# Autodesk Inventor assembly: St
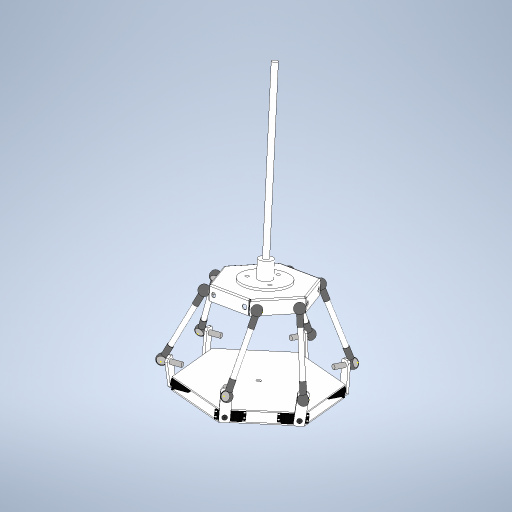
[picture p0: Inventor's stored thumbnail of the model, 512x512]
Saved by Autodesk Inventor 2023 (Build 270158000, 158)
## iProperties
Created: 2022-07-07
Part Number: St
Document SubType Name: Assembly
Designer: earls
Author: earls
## Documents named in this file (18)
- C:\Users\earls\Documents\stewart-platform\CAD\St.iam
- C:\Users\earls\Documents\stewart-platform\CAD\Bottom plate 2.5mm.ipt
- C:\Users\earls\Documents\stewart-platform\CAD\ServoMotor\Servo.ipt
- C:\Users\earls\Documents\stewart-platform\CAD\Servo arm.ipt
- C:\Users\earls\Documents\stewart-platform\CAD\Spherical joint\Part1.ipt
- C:\Users\earls\Documents\stewart-platform\CAD\Spherical joint\Part2.ipt
- C:\Users\earls\Documents\stewart-platform\CAD\Rod qty-6 Not hollow.ipt
- C:\Users\earls\Documents\stewart-platform\CAD\Moving platform.ipt
- C:\Users\earls\Documents\stewart-platform\CAD\Test flange.ipt
- C:\Users\earls\Documents\stewart-platform\CAD\Strut.ipt
- C:\Users\earls\Documents\stewart-platform\CAD\St\AIP\FEA\e0wa6g2m8.fins
- C:\Users\earls\Documents\stewart-platform\CAD\St\AIP\FEA\e0wa6g2m8.fsat
- C:\Users\earls\Documents\stewart-platform\CAD\St\AIP\FEA\e0wa6g2n4.ftes
- C:\Users\earls\Documents\stewart-platform\CAD\St\AIP\FEA\e0wa6g2n4.fwiz
- C:\Users\earls\Documents\stewart-platform\CAD\St\AIP\FEA\e0wa6g2u8.fmsh
- C:\Users\earls\Documents\stewart-platform\CAD\St\AIP\FEA\e0wa6g2v4.fres
- C:\Users\earls\Documents\stewart-platform\CAD\St\AIP\FEA\e0wa6g3cw.fmsh
- C:\Users\earls\Documents\stewart-platform\CAD\St\AIP\FEA\e0wa6g3cx.fres
## Components (47 placed, 9 different names)
1. Bottom plate 2.5mm:1 — Mate:4, Mate:5, Mate:6, Mate:7, Mate:8, Mate:9, Mate:10, Mate:11, Mate:12, Mate:13, Mate:14, Mate:15, Mate:16, Mate:17, Mate:18, Mate:20, Mate:21, Mate:22, Mate:23, Mate:24
2. Servo:1 — Mate:22, Mate:23, Mate:24, Rotational:6
3. Servo:3 — Mate:7, Mate:8, Mate:9, Rotational:3
4. Servo:4 — Mate:10, Mate:11, Mate:12, Mate:19, Rotational:2
5. Servo:5 — Mate:13, Mate:14, Mate:15, Rotational:4
6. Servo:6 — Mate:4, Mate:5, Mate:6, Rotational:1
7. Servo:7 — Mate:16, Mate:17, Mate:18, Rotational:5
8. Bottom plate 2.5mm:2 — Mate:19, Mate:20, Mate:21
9. Servo arm:1 — Rotational:2, Insert:1
10. Servo arm:2 — Rotational:4, Insert:4
11. Servo arm:3 — Rotational:5, Insert:3
12. Servo arm:4 — Rotational:6, Insert:6
13. Servo arm:5 — Rotational:1, Insert:5
14. Servo arm:6 — Rotational:3, Insert:2
15. Part1:1 — Ball:6, Mate:31, Mate:33
16. Part2:1 — Insert:3, Ball:4
17. Part1:2 — Ball:5, Mate:32, Mate:34
18. Part2:2 — Insert:2, Ball:5
19. Part1:3 — Ball:4, Mate:27, Mate:28
20. Part2:3 — Insert:6, Ball:1
21. Part1:4 — Ball:1, Mate:29, Mate:30
22. Part2:4 — Insert:1, Ball:6
23. Part1:5 — Ball:2, Rigid:1
24. Part2:5 — Insert:5, Ball:2
25. Part1:6 — Ball:3, Mate:25, Mate:26
26. Part2:6 — Insert:4, Ball:3
27. Rod qty-6 Not hollow:1 — Mate:31, Mate:33, Mate:38, Mate:46
28. Rod qty-6 Not hollow:2 — Mate:29, Mate:30, Mate:39, Mate:47
29. Rod qty-6 Not hollow:3 — Mate:32, Mate:34, Mate:36, Mate:37
30. Rod qty-6 Not hollow:4 — Rigid:1, Mate:40, Mate:43
31. Rod qty-6 Not hollow:5 — Mate:25, Mate:26, Mate:41, Mate:44
32. Rod qty-6 Not hollow:6 — Mate:27, Mate:28, Mate:42, Mate:45
33. Moving platform:1 — Insert:7, Insert:8, Insert:9, Insert:10, Insert:11, Insert:12, Mate:48, Mate:49, Mate:50, Mate:51
34. Part1:7 — Ball:7, Mate:38, Mate:46
35. Part2:7 — Insert:7, Ball:12
36. Part1:8 — Ball:10, Mate:42, Mate:45
37. Part2:8 — Insert:9, Ball:9
38. Part1:9 — Ball:9, Mate:41, Mate:44
39. Part2:9 — Insert:10, Ball:10
40. Part1:10 — Ball:11, Mate:40, Mate:43
41. Part2:10 — Insert:12, Ball:7
42. Part1:11 — Ball:8, Mate:36, Mate:37
43. Part2:11 — Insert:8, Ball:11
44. Part1:12 — Ball:12, Mate:39, Mate:47
45. Part2:12 — Insert:11, Ball:8
46. Test flange:1 — Mate:48, Mate:49, Mate:50, Mate:51, Rigid:2
47. Strut:1 — Rigid:2
## Relationships (79: Mate 47, Insert 12, BallJoint 12, RevoluteJoint 6, WeldJoint 2)
- Mate:4: Bottom plate 2.5mm:1 ↔ Servo:6
- Mate:5: Bottom plate 2.5mm:1 ↔ Servo:6
- Mate:6: Bottom plate 2.5mm:1 ↔ Servo:6
- Mate:7: Bottom plate 2.5mm:1 ↔ Servo:3
- Mate:8: Bottom plate 2.5mm:1 ↔ Servo:3
- Mate:9: Bottom plate 2.5mm:1 ↔ Servo:3
- Mate:10: Bottom plate 2.5mm:1 ↔ Servo:4
- Mate:11: Bottom plate 2.5mm:1 ↔ Servo:4
- Mate:12: Bottom plate 2.5mm:1 ↔ Servo:4
- Mate:13: Bottom plate 2.5mm:1 ↔ Servo:5
- Mate:14: Bottom plate 2.5mm:1 ↔ Servo:5
- Mate:15: Bottom plate 2.5mm:1 ↔ Servo:5
- Mate:16: Bottom plate 2.5mm:1 ↔ Servo:7
- Mate:17: Bottom plate 2.5mm:1 ↔ Servo:7
- Mate:18: Bottom plate 2.5mm:1 ↔ Servo:7
- Mate:19: Servo:4 ↔ Bottom plate 2.5mm:2
- Mate:20: Bottom plate 2.5mm:1 ↔ Bottom plate 2.5mm:2
- Mate:21: Bottom plate 2.5mm:1 ↔ Bottom plate 2.5mm:2
- Rotational:1 [RevoluteJoint]: Servo:6 ↔ Servo arm:5
- Rotational:2 [RevoluteJoint]: Servo:4 ↔ Servo arm:1
- Rotational:3 [RevoluteJoint]: Servo:3 ↔ Servo arm:6
- Rotational:4 [RevoluteJoint]: Servo:5 ↔ Servo arm:2
- Rotational:5 [RevoluteJoint]: Servo:7 ↔ Servo arm:3
- Mate:22: Bottom plate 2.5mm:1 ↔ Servo:1
- Mate:23: Bottom plate 2.5mm:1 ↔ Servo:1
- Mate:24: Bottom plate 2.5mm:1 ↔ Servo:1
- Rotational:6 [RevoluteJoint]: Servo:1 ↔ Servo arm:4
- Insert:1 (-3 mm): Servo arm:1 ↔ Part2:4
- Insert:2 (-3 mm): Servo arm:6 ↔ Part2:2
- Insert:3 (-3 mm): Servo arm:3 ↔ Part2:1
- Insert:4 (-3 mm): Servo arm:2 ↔ Part2:6
- Insert:5 (-3 mm): Servo arm:5 ↔ Part2:5
- Insert:6 (-3 mm): Servo arm:4 ↔ Part2:3
- Ball:1: Part2:3 ↔ Part1:4
- Ball:2: Part1:5 ↔ Part2:5
- Ball:3: Part1:6 ↔ Part2:6
- Ball:4: Part2:1 ↔ Part1:3
- Ball:5: Part1:2 ↔ Part2:2
- Ball:6: Part1:1 ↔ Part2:4
- Rigid:1 [WeldJoint]: Part1:5 ↔ Rod qty-6 Not hollow:4
- Mate:25: Part1:6 ↔ Rod qty-6 Not hollow:5
- Mate:26: Part1:6 ↔ Rod qty-6 Not hollow:5
- Mate:27: Part1:3 ↔ Rod qty-6 Not hollow:6
- Mate:28: Part1:3 ↔ Rod qty-6 Not hollow:6
- Mate:29: Part1:4 ↔ Rod qty-6 Not hollow:2
- Mate:30: Part1:4 ↔ Rod qty-6 Not hollow:2
- Mate:31: Part1:1 ↔ Rod qty-6 Not hollow:1
- Mate:32: Part1:2 ↔ Rod qty-6 Not hollow:3
- Mate:33: Part1:1 ↔ Rod qty-6 Not hollow:1
- Mate:34: Part1:2 ↔ Rod qty-6 Not hollow:3
- Insert:7 (-3 mm): Moving platform:1 ↔ Part2:7
- Insert:8 (-3 mm): Moving platform:1 ↔ Part2:11
- Insert:9 (-3 mm): Moving platform:1 ↔ Part2:8
- Insert:10 (-3 mm): Moving platform:1 ↔ Part2:9
- Insert:11 (-3 mm): Moving platform:1 ↔ Part2:12
- Insert:12 (-3 mm): Moving platform:1 ↔ Part2:10
- Ball:7: Part1:7 ↔ Part2:10
- Ball:8: Part1:11 ↔ Part2:12
- Ball:9: Part2:8 ↔ Part1:9
- Ball:10: Part1:8 ↔ Part2:9
- Ball:11: Part1:10 ↔ Part2:11
- Ball:12: Part2:7 ↔ Part1:12
- Mate:36: Rod qty-6 Not hollow:3 ↔ Part1:11
- Mate:37: Rod qty-6 Not hollow:3 ↔ Part1:11
- Mate:38: Rod qty-6 Not hollow:1 ↔ Part1:7
- Mate:39: Rod qty-6 Not hollow:2 ↔ Part1:12
- Mate:40: Rod qty-6 Not hollow:4 ↔ Part1:10
- Mate:41: Rod qty-6 Not hollow:5 ↔ Part1:9
- Mate:42: Rod qty-6 Not hollow:6 ↔ Part1:8
- Mate:43: Rod qty-6 Not hollow:4 ↔ Part1:10
- Mate:44: Rod qty-6 Not hollow:5 ↔ Part1:9
- Mate:45: Rod qty-6 Not hollow:6 ↔ Part1:8
- Mate:46: Rod qty-6 Not hollow:1 ↔ Part1:7
- Mate:47: Rod qty-6 Not hollow:2 ↔ Part1:12
- Mate:48: Moving platform:1 ↔ Test flange:1
- Mate:49: Moving platform:1 ↔ Test flange:1
- Mate:50: Moving platform:1 ↔ Test flange:1
- Mate:51: Moving platform:1 ↔ Test flange:1
- Rigid:2 [WeldJoint]: Test flange:1 ↔ Strut:1
## Named parameters: sa_0 = 39000, sa_1 = 25000
note: some values were not read from the file. Shown as the stored number, unit unknown: "sa_0", "sa_1".
